# Autodesk Inventor assembly: am-2256 4 in HiGrip Wheel
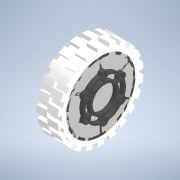
[picture p0: Inventor's stored thumbnail of the model, 180x180]
Saved by Autodesk Inventor 2020 (Build 240168000, 168)
## iProperties
Created: 2012-12-03
Part Number: am-2256 4 in HiGrip Wheel
Description: STEP AP214
Document SubType Name: Assembly
Designer: srini
Sending System: SolidWorks 2010
Preprocessor: SwSTEP 2.0
Title: 4 in HiGrip Wheel.STEP
Revision Number: ANY
## Documents named in this file (4)
- C:\Users\srini\Documents\FRC\2020\am-2256 4 in HiGrip Wheel.iam
- C:\Users\srini\Documents\FRC\2020\4in 2013 Hub.ipt
- C:\Users\srini\Documents\FRC\2020\4 in tread.ipt
- C:\Users\srini\Documents\FRC\2020\WheelMod4.ipt
## Components (3 placed, 3 different names)
1. 4in 2013 Hub_1
2. 4 in tread_2 — Flush:1
3. WheelMod4:1 — Flush:1
## Relationships (1: Flush 1)
- Flush:1: 4 in tread_2 ↔ WheelMod4:1
